# Autodesk Inventor assembly: s-assy-shooter_motor
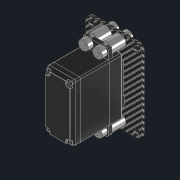
[picture p0: Inventor's stored thumbnail of the model, 180x180]
Saved by Autodesk Inventor 2022 (Build 260153000, 153)
## iProperties
Created: 2021-08-27
Part Number: s-assy-shooter_motor
Document SubType Name: Assembly
Designer: Yuta Kage
Author: Yuta Kage
## Documents named in this file (6)
- C:\Users\yuta0\Documents\GitHub\catchrobo_hardware\assy-shooter\s-assy-shooter_motor.iam
- C:\Users\yuta0\Documents\GitHub\catchrobo_hardware\assy-robot\MG_996R.iam
- C:\Users\yuta0\Documents\GitHub\catchrobo_hardware\assy-shooter\s_carbon_plate4.ipt
- C:\Users\yuta0\Documents\GitHub\catchrobo_hardware\assy-robot\ARF-410E.ipt
- C:\Users\yuta0\Documents\GitHub\catchrobo_hardware\assy-robot\CB4-6.ipt
- C:\Users\yuta0\Documents\GitHub\catchrobo_hardware\assy-robot\CBSTSR4-6.ipt
## Components (14 placed, 5 different names)
1. MG_996R:1 [sub-assembly] — メイト:18, メイト:19, メイト:20, メイト:22, メイト:24, メイト:25, メイト:35, メイト:50, メイト:51, メイト:52, メイト:53, メイト:54, メイト:55, メイト:56, メイト:57
2. s_carbon_plate4:1 — メイト:18, メイト:19, メイト:20, メイト:23, メイト:33, メイト:34, メイト:36, メイト:42, メイト:43, メイト:44, メイト:45, メイト:46, メイト:47, メイト:48, メイト:49
3. ARF-410E:2 — メイト:22, メイト:23
4. ARF-410E:3 — メイト:24, メイト:25
5. ARF-410E:4 — メイト:33, メイト:34
6. ARF-410E:5 — メイト:35, メイト:36
7. CBSTSR4-6:2 — メイト:42, メイト:43
8. CBSTSR4-6:3 — メイト:44, メイト:45
9. CB4-6:4 — メイト:46, メイト:47
10. CB4-6:5 — メイト:48, メイト:49
11. CB4-6:6 — メイト:50, メイト:51
12. CB4-6:7 — メイト:52, メイト:53
13. CB4-6:8 — メイト:54, メイト:55
14. CB4-6:9 — メイト:56, メイト:57
## Relationships (27: Mate 27)
- メイト:18 [Mate]: MG_996R:1 ↔ s_carbon_plate4:1
- メイト:19 [Mate]: MG_996R:1 ↔ s_carbon_plate4:1
- メイト:20 [Mate] (10 mm): MG_996R:1 ↔ s_carbon_plate4:1
- メイト:22 [Mate]: MG_996R:1 ↔ ARF-410E:2
- メイト:23 [Mate]: s_carbon_plate4:1 ↔ ARF-410E:2
- メイト:24 [Mate]: MG_996R:1 ↔ ARF-410E:3
- メイト:25 [Mate]: MG_996R:1 ↔ ARF-410E:3
- メイト:33 [Mate]: s_carbon_plate4:1 ↔ ARF-410E:4
- メイト:34 [Mate]: s_carbon_plate4:1 ↔ ARF-410E:4
- メイト:35 [Mate]: MG_996R:1 ↔ ARF-410E:5
- メイト:36 [Mate]: s_carbon_plate4:1 ↔ ARF-410E:5
- メイト:42 [Mate]: s_carbon_plate4:1 ↔ CBSTSR4-6:2
- メイト:43 [Mate]: s_carbon_plate4:1 ↔ CBSTSR4-6:2
- メイト:44 [Mate]: s_carbon_plate4:1 ↔ CBSTSR4-6:3
- メイト:45 [Mate]: s_carbon_plate4:1 ↔ CBSTSR4-6:3
- メイト:46 [Mate]: s_carbon_plate4:1 ↔ CB4-6:4
- メイト:47 [Mate]: s_carbon_plate4:1 ↔ CB4-6:4
- メイト:48 [Mate]: s_carbon_plate4:1 ↔ CB4-6:5
- メイト:49 [Mate]: s_carbon_plate4:1 ↔ CB4-6:5
- メイト:50 [Mate]: MG_996R:1 ↔ CB4-6:6
- メイト:51 [Mate]: MG_996R:1 ↔ CB4-6:6
- メイト:52 [Mate]: MG_996R:1 ↔ CB4-6:7
- メイト:53 [Mate]: MG_996R:1 ↔ CB4-6:7
- メイト:54 [Mate]: MG_996R:1 ↔ CB4-6:8
- メイト:55 [Mate]: MG_996R:1 ↔ CB4-6:8
- メイト:56 [Mate]: MG_996R:1 ↔ CB4-6:9
- メイト:57 [Mate]: MG_996R:1 ↔ CB4-6:9
